# Autodesk Inventor assembly: ADSK-MH-10010
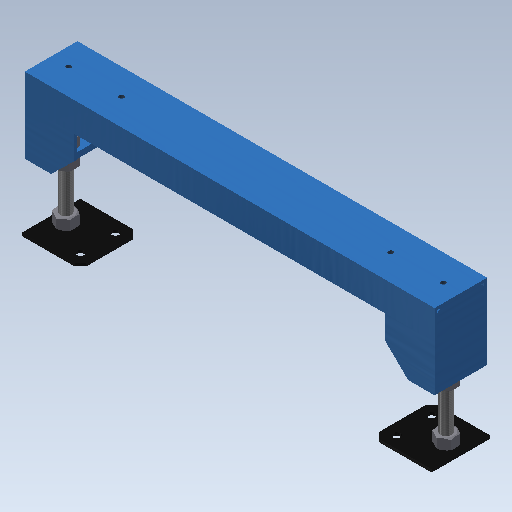
[picture p0: Inventor's stored thumbnail of the model, 512x512]
Saved by Autodesk Inventor 2021.1 (Build 251245010, 245A)
## iProperties
Created: 2008-03-10
Part Number: ADSK-MH-10010
Document SubType Name: Assembly
Designer: R.O'mahony
Description: Conveyor Outer Beam
Engineer: Demir Ali
Checked By: Demir Ali
Company: Autodesk Ltd
Author: R.O'mahony
Keywords: Roller Conveyor
Revision Number: A
## Documents named in this file (6)
- C:\Users\peter\source\repos\InventorDA-FLC\Dataset\Discharge Conveyor\ADSK-MH-10010.iam
- C:\Users\peter\source\repos\InventorDA-FLC\Dataset\Discharge Conveyor\ADSK-MH-10045.ipt
- C:\Users\peter\source\repos\InventorDA-FLC\Dataset\Discharge Conveyor\ADSK-MH-10043.ipt
- C:\Users\peter\source\repos\InventorDA-FLC\Dataset\Discharge Conveyor\ISO 4034 - M20ISO.ipt
- C:\Users\peter\source\repos\InventorDA-FLC\Dataset\Discharge Conveyor\ADSK-MH-10011.ipt
- C:\Users\peter\source\repos\InventorDA-FLC\Dataset\Discharge Conveyor\ADSK-MH-10012.iam
## Components (11 placed, 5 different names)
1. Leg Top Support — Rigid:1, Rigid:2
2. ADSK-MH-10045:1 — Flush:3, Mate:3, Mate:4, Angle:1, Rigid:1
3. ADSK-MH-10045:2 — Flush:4, Mate:5, Mate:6, Angle:2, Rigid:2
4. ADSK-MH-10043:1 — Flush:3, Mate:3, Mate:4, Insert:2, Insert:3
5. ADSK-MH-10043:2 — Flush:4, Mate:5, Mate:6, Insert:1, Insert:4
6. ISO 4034 M20:1 — Insert:1, Insert:6
7. ISO 4034 M20:2 — Insert:2
8. ISO 4034 M20:3 — Insert:4
9. ISO 4034 M20:4 — Insert:3
10. ADSK-MH-10012:1 [sub-assembly] — Insert:6, Angle:2
11. ADSK-MH-10012:2 [sub-assembly] — Angle:1
## Relationships (16: Insert 6, Mate 4, Flush 2, Angle 2, WeldJoint 2)
- Flush:3: ADSK-MH-10045:1 ↔ ADSK-MH-10043:1
- Mate:3: ADSK-MH-10045:1 ↔ ADSK-MH-10043:1
- Mate:4: ADSK-MH-10045:1 ↔ ADSK-MH-10043:1
- Flush:4: ADSK-MH-10045:2 ↔ ADSK-MH-10043:2
- Mate:5: ADSK-MH-10045:2 ↔ ADSK-MH-10043:2
- Mate:6: ADSK-MH-10045:2 ↔ ADSK-MH-10043:2
- Insert:2: ADSK-MH-10043:1 ↔ ISO 4034 M20:2
- Insert:3: ADSK-MH-10043:1 ↔ ISO 4034 M20:4
- Insert:4: ADSK-MH-10043:2 ↔ ISO 4034 M20:3
- [Insert] (-20 mm): ISO 4034 M20:2 ↔ ADSK-MH-10012:2
- Angle:1 (0 deg): ADSK-MH-10045:1 ↔ ADSK-MH-10012:2
- Insert:6 (-20 mm): ISO 4034 M20:1 ↔ ADSK-MH-10012:1
- Angle:2 (180 deg): ADSK-MH-10045:2 ↔ ADSK-MH-10012:1
- Insert:1: ADSK-MH-10043:2 ↔ ISO 4034 M20:1
- Rigid:1 [WeldJoint]: Leg Top Support ↔ ADSK-MH-10045:1
- Rigid:2 [WeldJoint]: Leg Top Support ↔ ADSK-MH-10045:2
